# Autodesk Inventor assembly: LINK4
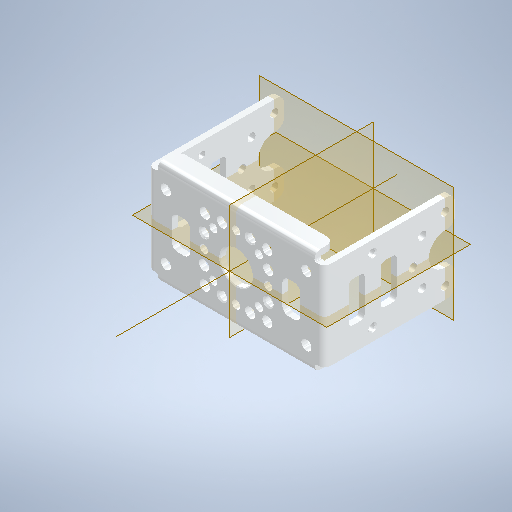
[picture p0: Inventor's stored thumbnail of the model, 512x512]
Saved by Autodesk Inventor 2026.1 (Build 301233020, 233B)
## iProperties
Created: 2025-10-15
Part Number: LINK4
Document SubType Name: Assembly
Designer: wlgns
Author: wlgns
## Documents named in this file (2)
- C:\Users\wlgns\Desktop\project\ARA Project\ARA_CAD_model\ARA_v2\LINK4.iam
- C:\Users\wlgns\Desktop\project\ARA Project\ARA_CAD_model\ARA_v2\fr07_h101 - mx28 frame.ipt
## Components (1 placed, 1 different names)
1. fr07_h101 - mx28 frame:1 — 플러쉬:1, 메이트:2
## Relationships (4: Mate 3, Flush 1)
- 플러쉬:1 [Flush] (-2.5 mm): fr07_h101 - mx28 frame:1
- 메이트:1 [Mate]
- 메이트:2 [Mate]: fr07_h101 - mx28 frame:1
- 메이트:3 [Mate]
